# Autodesk Inventor assembly: CameraSystem
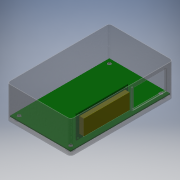
[picture p0: Inventor's stored thumbnail of the model, 180x180]
Saved by Autodesk Inventor 2016 (Build 200138000, 138)
## iProperties
Created: 2018-10-10
Part Number: CameraSystem
Document SubType Name: Assembly
Designer: vtolenti89
Author: vtolenti89
## Documents named in this file (4)
- C:\Users\vtolenti89\Documents\Projects\Kicad\Projects\CameraSystem\Mechanics\CameraSystem.iam
- C:\Users\vtolenti89\Documents\DisplayWithI2c.ipt
- C:\Users\vtolenti89\Documents\HousingBottom.ipt
- C:\Users\vtolenti89\Documents\Projects\Kicad\Projects\CameraSystem\Mechanics\PCBBase.ipt
## Components (3 placed, 3 different names)
1. DisplayWithI2c:1 — Mate:2, Mate:3, Flush:3
2. HousingBottom:1 — Flush:1, Flush:2, Mate:2, Flush:3
3. PCBBase:1 — Flush:2, Mate:3
## Relationships (5: Flush 3, Mate 2)
- Flush:1: HousingBottom:1
- Flush:2: HousingBottom:1 ↔ PCBBase:1
- Mate:2 (15 mm): DisplayWithI2c:1 ↔ HousingBottom:1
- Mate:3 (5 mm): DisplayWithI2c:1 ↔ PCBBase:1
- Flush:3: DisplayWithI2c:1 ↔ HousingBottom:1
